# Autodesk Inventor assembly: Viewpoint
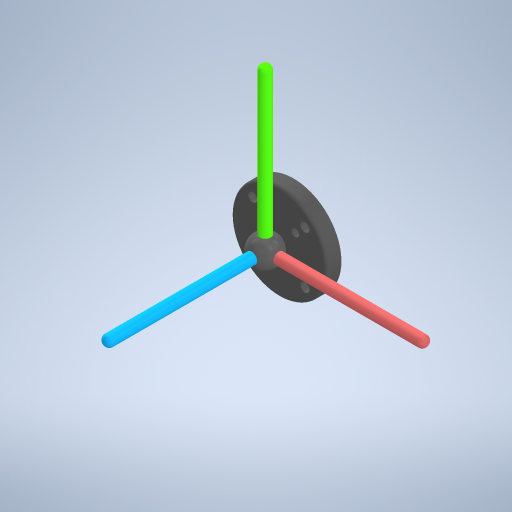
[picture p0: Inventor's stored thumbnail of the model, 512x512]
Saved by Autodesk Inventor 2023 (Build 270158000, 158)
## iProperties
Created: 2022-12-18
Part Number: Viewpoint
Document SubType Name: Assembly
Designer: romanp
Author: romanp
## Documents named in this file (3)
- C:\Users\romanp\Desktop\Viewpoint.iam
- C:\Users\romanp\Desktop\Part_Top.ipt
- C:\Users\romanp\Desktop\Viewpoint_T1.ipt
## Components (2 placed, 2 different names)
1. Part_Top:1 — Insert:1, Insert:2
2. Viewpoint_T1:1 — Insert:1, Insert:2
## Relationships (2: Insert 2)
- Insert:1: Part_Top:1 ↔ Viewpoint_T1:1
- Insert:2: Part_Top:1 ↔ Viewpoint_T1:1
